# Autodesk Inventor assembly: Tool_post
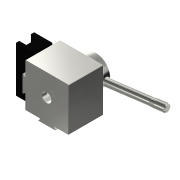
[picture p0: Inventor's stored thumbnail of the model, 180x180]
Saved by Autodesk Inventor 2016 (Build 200138000, 138)
## iProperties
Created: 2020-10-21
Part Number: Tool_post
Document SubType Name: Assembly
Designer: extract
Author: extract
## Documents named in this file (6)
- D:\GDrive\Proyecto_Torno\Tool_post\Tool_post.iam
- D:\GDrive\Proyecto_Torno\Tool_post\Tool Post Block.ipt
- D:\GDrive\Proyecto_Torno\Tool_post\Midle.ipt
- D:\GDrive\Proyecto_Torno\Tool_post\Top.ipt
- D:\GDrive\Proyecto_Torno\Tool_post\Handbar.ipt
- D:\GDrive\Proyecto_Torno\Tool_post\Holder.iam
## Components (5 placed, 5 different names)
1. Tool Post Block:1 — Cylindrical:4, Mate:1, Mate:4, Insert:1
2. Midle:1 — Cylindrical:2, Cylindrical:3, Cylindrical:4, Insert:1
3. Top:1 — Cylindrical:2
4. Handbar:1 — Cylindrical:3
5. Holder:1 [sub-assembly] — Mate:1, Mate:4
## Relationships (6: CylindricalJoint 3, Mate 2, Insert 1)
- Cylindrical:2: Midle:1 ↔ Top:1
- Cylindrical:3: Midle:1 ↔ Handbar:1
- Cylindrical:4: Tool Post Block:1 ↔ Midle:1
- Mate:1: Tool Post Block:1 ↔ Holder:1
- Mate:4: Tool Post Block:1 ↔ Holder:1
- Insert:1: Tool Post Block:1 ↔ Midle:1
